# Autodesk Inventor assembly: SampleHolder
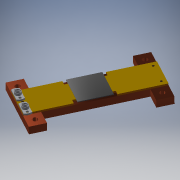
[picture p0: Inventor's stored thumbnail of the model, 180x180]
Saved by Autodesk Inventor 2017 SP1 (Build 210196100, 196)
## iProperties
Created: 2017-02-03
Part Number: SampleHolder
Document SubType Name: Assembly
Designer: Alex
Author: Alex
## Documents named in this file (5)
- C:\Users\Alex\Documents\git\CPWResonator\Inventor\Assemblies\Sample holder 20x20.iam
- C:\Users\Alex\Documents\git\CPWResonator\Inventor\Mount\Mount base.ipt
- C:\Users\Alex\Documents\git\CPWResonator\Inventor\PCBs\PCB blank 20x20.ipt
- C:\Users\Alex\Documents\git\CPWResonator\Inventor\Chips\Chip blank 20x20.ipt
- C:\Users\Alex\Documents\git\CPWResonator\Inventor\PCBs\SMP connector vertical.ipt
## Components (5 placed, 4 different names)
1. Mount base:1 — Mate:1, Mate:4, Angle:2
2. PCB blank 20x20:1 — Mate:1, Mate:2, Angle:1, Mate:4, Mate:5, Angle:2, Mate:6, Mate:7, Flush:1, Flush:2
3. Chip blank 20x20:1 — Mate:2, Mate:3, Angle:1
4. SMP connector vertical:1 — Mate:6, Flush:2
5. SMP connector vertical:2 — Mate:7, Flush:1
## Relationships (11: Mate 7, Angle 2, Flush 2)
- Mate:1: Mount base:1 ↔ PCB blank 20x20:1
- Mate:2: PCB blank 20x20:1 ↔ Chip blank 20x20:1
- Mate:3: Chip blank 20x20:1
- Angle:1 (0 deg): PCB blank 20x20:1 ↔ Chip blank 20x20:1
- Mate:4: Mount base:1 ↔ PCB blank 20x20:1
- Mate:5: PCB blank 20x20:1
- Angle:2 (0 deg): Mount base:1 ↔ PCB blank 20x20:1
- Mate:6: PCB blank 20x20:1 ↔ SMP connector vertical:1
- Mate:7: PCB blank 20x20:1 ↔ SMP connector vertical:2
- Flush:1: PCB blank 20x20:1 ↔ SMP connector vertical:2
- Flush:2: PCB blank 20x20:1 ↔ SMP connector vertical:1
